# Autodesk Inventor assembly: SCR3_15_100
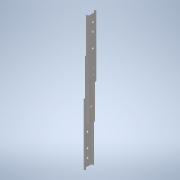
[picture p0: Inventor's stored thumbnail of the model, 180x180]
Saved by Autodesk Inventor 2022.3 (Build 263350000, 350)
## iProperties
Created: 2022-04-11
Part Number: SCR3_15_100
Document SubType Name: Assembly
Designer: YusukeKunita
Author: YusukeKunita
## Documents named in this file (3)
- C:\Users\YusukeKunita\Documents\GrabCAD\NHK2022\BasicParts\SlideRail\SCR3_15_100\SCR3_15_100.iam
- C:\Users\YusukeKunita\Documents\GrabCAD\NHK2022\BasicParts\SlideRail\SCR3_15_100\SCR3_15_100A_outer_SCR3-15-100_.ipt
- C:\Users\YusukeKunita\Documents\GrabCAD\NHK2022\BasicParts\SlideRail\SCR3_15_100\SCR3_15_100A_inner_SCR3-15-100.ipt
## Components (3 placed, 2 different names)
1. SCR3_15_100A_outer_SCR3-15-100_:3
2. SCR3_15_100A_outer_SCR3-15-100_:4
3. SCR3_15_100A_inner_SCR3-15-100:1
## Relationships (2: TranslationJoint 2)
- [TranslationJoint] (3.45 mm): SCR3_15_100A_outer_SCR3-15-100_:4 ↔ SCR3_15_100A_inner_SCR3-15-100:1
- [TranslationJoint] (3.45 mm): SCR3_15_100A_outer_SCR3-15-100_:3 ↔ SCR3_15_100A_inner_SCR3-15-100:1
## Named parameters: d892_d4 = 0 mm, d893_d5 = 62.5 mm, d894_d6 = 0 mm, d895_d7 = 62.5 mm, d896_Distance1_3 = 3.45 mm, d897_Distance2_3 = 3.45 mm, d898_d0 = 3.45 mm, d899_d1 = 0.621 mm, d901_d3 = 0 mm
